# Autodesk Inventor assembly: ParallelMechanismus_Driven_Assembly_v2.1_Nadellager
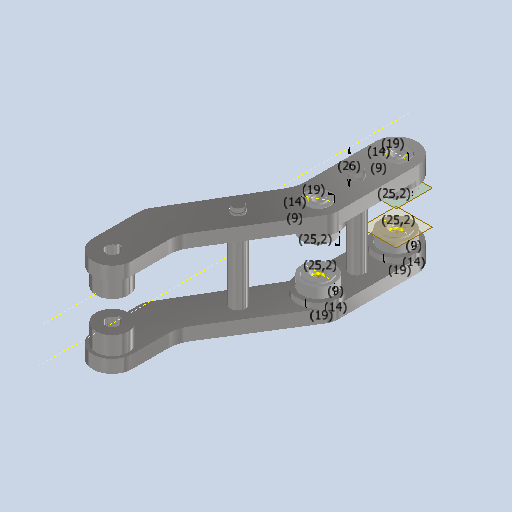
[picture p0: Inventor's stored thumbnail of the model, 512x512]
Saved by Autodesk Inventor 2022 (Build 260153000, 153)
## iProperties
Created: 2022-07-21
Part Number: ParallelMechanismus_Driven_Assembly_v2.1_Nadellager
Document SubType Name: Assembly
Designer: alexw
ParallelMecha_Contact_Dist: 26,000 mm
Author: alexw
## Documents named in this file (8)
- C:\Users\alexw\Documents\Inventor\Projects\03_CurrentProjects\MasterThesis\Parallelsystem_DaVinci_CAD\ParallelMechanismus_Driven_Assembly_v2.1_Nadellager.iam
- C:\Users\alexw\Documents\Inventor\Projects\03_CurrentProjects\MasterThesis\Parallelsystem_DaVinci_CAD\ParallelSystem_ProximalPart_Driven_v2.1_AxialNadellager.ipt
- C:\Users\alexw\Documents\Inventor\Projects\03_CurrentProjects\MasterThesis\Parallelsystem_DaVinci_CAD\Downloads\SKF_NKX 10 ZTN\SKF_NKX 10 ZTN.iam
- C:\Users\alexw\Documents\Inventor\Projects\03_CurrentProjects\MasterThesis\Parallelsystem_DaVinci_CAD\ParallelSystem_ProximalPart_Querstreben_v2.ipt
- C:\Users\alexw\Documents\Inventor\Projects\03_CurrentProjects\MasterThesis\Parallelsystem_DaVinci_CAD\ParallelSystem_ProximalPart_Driven_Counterpart_v2.1_AxialNadellager.ipt
- C:\Users\alexw\Documents\Inventor\Projects\03_CurrentProjects\MasterThesis\Parallelsystem_DaVinci_CAD\Downloads\SKF_NKX 10 ZTN\SKF_IR 7X10X16.ipt
- C:\Users\alexw\Documents\Inventor\Content Center Files\R2022\de-DE\ISO 7090\ISO 7090 - 5 - 140 HV(1).ipt
- C:\Users\alexw\Documents\Inventor\Content Center Files\R2022\de-DE\ISO 4017(1)\ISO 4017 - M5 x 10 - ISO.ipt
## Components (20 placed, 7 different names)
1. ParallelSystem_ProximalPart_Driven_v2.1_AxialNadellager:1 — Fluchtend:1, Fluchtend:2, Fluchtend:3, Passend:10, Passend:11, Passend:12, Passend:23, Einfügen:3, Einfügen:4, Passend:47, Passend:49
2. SKF_NKX 10 ZTN:1 [sub-assembly] — Passend:10, Passend:42, Fluchtend:4
3. SKF_NKX 10 ZTN:2 [sub-assembly] — Passend:11, Passend:12, Passend:45, Fluchtend:6, Fluchtend:8
4. ParallelSystem_ProximalPart_Querstreben_v2:1 — Einfügen:4, Einfügen:5, Passend:48, Passend:50, Passend:56, Passend:58
5. ParallelSystem_ProximalPart_Querstreben_v2:2 — Einfügen:3, Einfügen:6, Passend:46, Passend:52, Passend:54, Passend:60
6. ParallelSystem_ProximalPart_Driven_Counterpart_v2.1_AxialNadellager:1 — Passend:23, Passend:32, Passend:33, Passend:34, Passend:35, Einfügen:5, Einfügen:6, Passend:51, Passend:53
7. SKF_NKX 10 ZTN:3 [sub-assembly] — Passend:34, Passend:35, Passend:44, Fluchtend:7, Fluchtend:9
8. SKF_NKX 10 ZTN:4 [sub-assembly] — Passend:32, Passend:33, Passend:43, Fluchtend:5
9. SKF_IR 7X10X16:1 — Passend:42, Fluchtend:4
10. SKF_IR 7X10X16:2 — Passend:43, Fluchtend:5
11. SKF_IR 7X10X16:3 — Passend:45, Fluchtend:6
12. SKF_IR 7X10X16:4 — Passend:44, Fluchtend:7
13. ISO 7090 5 - 140 HV:1 — Passend:46, Passend:47, Passend:61
14. ISO 7090 5 - 140 HV:2 — Passend:48, Passend:49, Passend:59
15. ISO 7090 5 - 140 HV:3 — Passend:50, Passend:51, Passend:57
16. ISO 7090 5 - 140 HV:4 — Passend:52, Passend:53, Passend:55
17. ISO 4017 M5 x 10:1 — Passend:54, Passend:55
18. ISO 4017 M5 x 10:2 — Passend:56, Passend:57
19. ISO 4017 M5 x 10:3 — Passend:58, Passend:59
20. ISO 4017 M5 x 10:4 — Passend:60, Passend:61
## Relationships (41: Mate 28, Flush 9, Insert 4)
- Fluchtend:1 [Flush]: ParallelSystem_ProximalPart_Driven_v2.1_AxialNadellager:1
- Fluchtend:2 [Flush]: ParallelSystem_ProximalPart_Driven_v2.1_AxialNadellager:1
- Fluchtend:3 [Flush]: ParallelSystem_ProximalPart_Driven_v2.1_AxialNadellager:1
- Passend:10 [Mate]: ParallelSystem_ProximalPart_Driven_v2.1_AxialNadellager:1 ↔ SKF_NKX 10 ZTN:1
- Passend:11 [Mate]: ParallelSystem_ProximalPart_Driven_v2.1_AxialNadellager:1 ↔ SKF_NKX 10 ZTN:2
- Passend:12 [Mate]: ParallelSystem_ProximalPart_Driven_v2.1_AxialNadellager:1 ↔ SKF_NKX 10 ZTN:2
- Passend:23 [Mate]: ParallelSystem_ProximalPart_Driven_v2.1_AxialNadellager:1 ↔ ParallelSystem_ProximalPart_Driven_Counterpart_v2.1_AxialNadellager:1
- Passend:32 [Mate]: ParallelSystem_ProximalPart_Driven_Counterpart_v2.1_AxialNadellager:1 ↔ SKF_NKX 10 ZTN:4
- Passend:33 [Mate]: ParallelSystem_ProximalPart_Driven_Counterpart_v2.1_AxialNadellager:1 ↔ SKF_NKX 10 ZTN:4
- Passend:34 [Mate]: ParallelSystem_ProximalPart_Driven_Counterpart_v2.1_AxialNadellager:1 ↔ SKF_NKX 10 ZTN:3
- Passend:35 [Mate]: ParallelSystem_ProximalPart_Driven_Counterpart_v2.1_AxialNadellager:1 ↔ SKF_NKX 10 ZTN:3
- Passend:42 [Mate]: SKF_NKX 10 ZTN:1 ↔ SKF_IR 7X10X16:1
- Fluchtend:4 [Flush]: SKF_NKX 10 ZTN:1 ↔ SKF_IR 7X10X16:1
- Passend:43 [Mate]: SKF_NKX 10 ZTN:4 ↔ SKF_IR 7X10X16:2
- Fluchtend:5 [Flush]: SKF_NKX 10 ZTN:4 ↔ SKF_IR 7X10X16:2
- Passend:44 [Mate]: SKF_NKX 10 ZTN:3 ↔ SKF_IR 7X10X16:4
- Passend:45 [Mate]: SKF_NKX 10 ZTN:2 ↔ SKF_IR 7X10X16:3
- Fluchtend:6 [Flush]: SKF_NKX 10 ZTN:2 ↔ SKF_IR 7X10X16:3
- Fluchtend:7 [Flush]: SKF_NKX 10 ZTN:3 ↔ SKF_IR 7X10X16:4
- Fluchtend:8 [Flush]: SKF_NKX 10 ZTN:2
- Fluchtend:9 [Flush]: SKF_NKX 10 ZTN:3
- Einfügen:3 [Insert]: ParallelSystem_ProximalPart_Driven_v2.1_AxialNadellager:1 ↔ ParallelSystem_ProximalPart_Querstreben_v2:2
- Einfügen:4 [Insert]: ParallelSystem_ProximalPart_Driven_v2.1_AxialNadellager:1 ↔ ParallelSystem_ProximalPart_Querstreben_v2:1
- Einfügen:5 [Insert]: ParallelSystem_ProximalPart_Querstreben_v2:1 ↔ ParallelSystem_ProximalPart_Driven_Counterpart_v2.1_AxialNadellager:1
- Einfügen:6 [Insert]: ParallelSystem_ProximalPart_Querstreben_v2:2 ↔ ParallelSystem_ProximalPart_Driven_Counterpart_v2.1_AxialNadellager:1
- Passend:46 [Mate]: ParallelSystem_ProximalPart_Querstreben_v2:2 ↔ ISO 7090 5 - 140 HV:1
- Passend:47 [Mate]: ParallelSystem_ProximalPart_Driven_v2.1_AxialNadellager:1 ↔ ISO 7090 5 - 140 HV:1
- Passend:48 [Mate]: ParallelSystem_ProximalPart_Querstreben_v2:1 ↔ ISO 7090 5 - 140 HV:2
- Passend:49 [Mate]: ParallelSystem_ProximalPart_Driven_v2.1_AxialNadellager:1 ↔ ISO 7090 5 - 140 HV:2
- Passend:50 [Mate]: ParallelSystem_ProximalPart_Querstreben_v2:1 ↔ ISO 7090 5 - 140 HV:3
- Passend:51 [Mate]: ParallelSystem_ProximalPart_Driven_Counterpart_v2.1_AxialNadellager:1 ↔ ISO 7090 5 - 140 HV:3
- Passend:52 [Mate]: ParallelSystem_ProximalPart_Querstreben_v2:2 ↔ ISO 7090 5 - 140 HV:4
- Passend:53 [Mate]: ParallelSystem_ProximalPart_Driven_Counterpart_v2.1_AxialNadellager:1 ↔ ISO 7090 5 - 140 HV:4
- Passend:54 [Mate]: ParallelSystem_ProximalPart_Querstreben_v2:2 ↔ ISO 4017 M5 x 10:1
- Passend:55 [Mate]: ISO 7090 5 - 140 HV:4 ↔ ISO 4017 M5 x 10:1
- Passend:56 [Mate]: ParallelSystem_ProximalPart_Querstreben_v2:1 ↔ ISO 4017 M5 x 10:2
- Passend:57 [Mate]: ISO 7090 5 - 140 HV:3 ↔ ISO 4017 M5 x 10:2
- Passend:58 [Mate]: ParallelSystem_ProximalPart_Querstreben_v2:1 ↔ ISO 4017 M5 x 10:3
- Passend:59 [Mate]: ISO 7090 5 - 140 HV:2 ↔ ISO 4017 M5 x 10:3
- Passend:60 [Mate]: ParallelSystem_ProximalPart_Querstreben_v2:2 ↔ ISO 4017 M5 x 10:4
- Passend:61 [Mate]: ISO 7090 5 - 140 HV:1 ↔ ISO 4017 M5 x 10:4
## Named parameters: ParallelMecha_Contact_Dist = 26 mm
